# Autodesk Inventor assembly: EmergencyWake
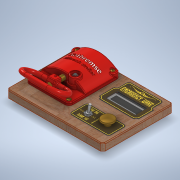
[picture p0: Inventor's stored thumbnail of the model, 180x180]
Saved by Autodesk Inventor 2020 (Build 240168000, 168)
## iProperties
Created: 2020-06-21
Part Number: EmergencyWake
Document SubType Name: Assembly
Designer: Johannes
Author: Johannes
## Documents named in this file (17)
- D:\Dokumente\Projekte\EmergencyWake\CAD\Inventor\EmergencyWake.iam
- D:\Dokumente\Projekte\EmergencyWake\CAD\Inventor\EW_Holzplatte.ipt
- D:\Dokumente\Projekte\EmergencyWake\CAD\Inventor\EW_Display.ipt
- D:\Dokumente\Projekte\EmergencyWake\CAD\Inventor\EW_MessingplatteBedienelemente.ipt
- D:\Dokumente\Projekte\EmergencyWake\CAD\Inventor\EW_MessingplatteUhrzeit.ipt
- D:\Dokumente\Projekte\EmergencyWake\CAD\Inventor\EW_NotbremseGehaeuse.ipt
- D:\Dokumente\Projekte\EmergencyWake\CAD\Inventor\EW_NotbremseHebel.ipt
- D:\Dokumente\Projekte\EmergencyWake\CAD\Inventor\EW_Plexiglas.ipt
- D:\Dokumente\Projekte\EmergencyWake\CAD\Inventor\ToggleSwitchKN3.ipt
- D:\Dokumente\Projekte\EmergencyWake\CAD\Inventor\Board\EmergencyWake.iam
- D:\Dokumente\Projekte\EmergencyWake\CAD\Inventor\DIN964_M5x16_Messing.ipt
- D:\Dokumente\Projekte\EmergencyWake\CAD\Inventor\RotaryEncoder\RotaryEncoder_ALPS_STEC11B.iam
- D:\Dokumente\Projekte\EmergencyWake\CAD\Inventor\EW_Drehknopf.ipt
- D:\Dokumente\Projekte\EmergencyWake\CAD\Inventor\EW_KunststoffEinsatz.ipt
- D:\Dokumente\Projekte\EmergencyWake\CAD\Inventor\EW_HebelAchse.ipt
- D:\Dokumente\Projekte\EmergencyWake\CAD\Inventor\D_090W_06_10mm.ipt
- D:\Dokumente\Projekte\EmergencyWake\CAD\Inventor\EW_Achsenabschluss.ipt
## Components (19 placed, 16 different names)
1. EW_Holzplatte:1 — Passend:1, Passend:2, Passend:3, Fluchtend:1, Fluchtend:2, Fluchtend:3, Fluchtend:4, Fluchtend:5, Passend:5, Passend:6, Fluchtend:6, Passend:8, Passend:9, Passend:10, Passend:11, Passend:12, Winkel:1, Einfügen:6, Winkel:2
2. EW_Display:1 — Passend:7, Fluchtend:7, Fluchtend:8
3. EW_MessingplatteBedienelemente:1 — Passend:2, Fluchtend:5, Passend:4, Einfügen:7
4. EW_MessingplatteUhrzeit:1 — Passend:3, Fluchtend:3, Fluchtend:4, Passend:4
5. EW_NotbremseGehaeuse:1 — Passend:1, Fluchtend:1, Fluchtend:2, Einfügen:2, Einfügen:3, Einfügen:4, Einfügen:5, Einfügen:8, Winkel:3, Winkel:4
6. EW_NotbremseHebel:1 — Einfügen:9, Winkel:4
7. EW_Plexiglas:1 — Passend:5, Passend:6, Fluchtend:6
8. ToggleSwitchKN3:1 — Passend:11, Passend:12, Winkel:1
9. EmergencyWake:1 [sub-assembly] — Passend:7, Fluchtend:7, Fluchtend:8, Passend:8, Passend:9, Passend:10
10. DIN EN ISO 2010 M5x16:1 — Einfügen:2
11. DIN EN ISO 2010 M5x16:2 — Einfügen:3
12. DIN EN ISO 2010 M5x16:3 — Einfügen:5
13. DIN EN ISO 2010 M5x16:4 — Einfügen:4
14. RotaryEncoder_ALPS_STEC11B:1 [sub-assembly] — Einfügen:6, Winkel:2
15. EW_Drehknopf:1 — Einfügen:7
16. EW_KunststoffEinsatz:1 — Einfügen:8, Winkel:3, Passend:13, Passend:14, Passend:16
17. EW_HebelAchse:1 — Passend:13, Passend:14, Einfügen:9, Passend:15, Einfügen:10
18. D_090W_06_10mm:1 — Passend:15, Passend:16
19. EW_Achsenabschluss:1 — Einfügen:10
## Relationships (37: Mate 16, Insert 9, Flush 8, Angle 4)
- Passend:1 [Mate]: EW_Holzplatte:1 ↔ EW_NotbremseGehaeuse:1
- Passend:2 [Mate]: EW_Holzplatte:1 ↔ EW_MessingplatteBedienelemente:1
- Passend:3 [Mate]: EW_Holzplatte:1 ↔ EW_MessingplatteUhrzeit:1
- Fluchtend:1 [Flush] (-10 mm): EW_Holzplatte:1 ↔ EW_NotbremseGehaeuse:1
- Fluchtend:2 [Flush] (-10 mm): EW_Holzplatte:1 ↔ EW_NotbremseGehaeuse:1
- Fluchtend:3 [Flush] (10 mm): EW_Holzplatte:1 ↔ EW_MessingplatteUhrzeit:1
- Fluchtend:4 [Flush] (10 mm): EW_Holzplatte:1 ↔ EW_MessingplatteUhrzeit:1
- Fluchtend:5 [Flush] (10 mm): EW_Holzplatte:1 ↔ EW_MessingplatteBedienelemente:1
- Passend:4 [Mate] (25 mm): EW_MessingplatteBedienelemente:1 ↔ EW_MessingplatteUhrzeit:1
- Passend:5 [Mate]: EW_Holzplatte:1 ↔ EW_Plexiglas:1
- Passend:6 [Mate]: EW_Holzplatte:1 ↔ EW_Plexiglas:1
- Fluchtend:6 [Flush]: EW_Holzplatte:1 ↔ EW_Plexiglas:1
- Passend:7 [Mate] (1 mm): EW_Display:1 ↔ EmergencyWake:1
- Fluchtend:7 [Flush] (0.9 mm): EW_Display:1 ↔ EmergencyWake:1
- Fluchtend:8 [Flush] (10 mm): EW_Display:1 ↔ EmergencyWake:1
- Passend:8 [Mate]: EW_Holzplatte:1 ↔ EmergencyWake:1
- Passend:9 [Mate] (15 mm): EW_Holzplatte:1 ↔ EmergencyWake:1
- Passend:10 [Mate] (2.5 mm): EW_Holzplatte:1 ↔ EmergencyWake:1
- Passend:11 [Mate]: EW_Holzplatte:1 ↔ ToggleSwitchKN3:1
- Passend:12 [Mate]: EW_Holzplatte:1 ↔ ToggleSwitchKN3:1
- Winkel:1 [Angle] (0 deg): EW_Holzplatte:1 ↔ ToggleSwitchKN3:1
- Einfügen:2 [Insert]: EW_NotbremseGehaeuse:1 ↔ DIN EN ISO 2010 M5x16:1
- Einfügen:3 [Insert]: EW_NotbremseGehaeuse:1 ↔ DIN EN ISO 2010 M5x16:2
- Einfügen:4 [Insert]: EW_NotbremseGehaeuse:1 ↔ DIN EN ISO 2010 M5x16:4
- Einfügen:5 [Insert]: EW_NotbremseGehaeuse:1 ↔ DIN EN ISO 2010 M5x16:3
- Einfügen:6 [Insert]: EW_Holzplatte:1 ↔ RotaryEncoder_ALPS_STEC11B:1
- Winkel:2 [Angle] (0 deg): EW_Holzplatte:1 ↔ RotaryEncoder_ALPS_STEC11B:1
- Einfügen:7 [Insert] (1 mm): EW_MessingplatteBedienelemente:1 ↔ EW_Drehknopf:1
- Einfügen:8 [Insert]: EW_NotbremseGehaeuse:1 ↔ EW_KunststoffEinsatz:1
- Winkel:3 [Angle] (0 deg): EW_NotbremseGehaeuse:1 ↔ EW_KunststoffEinsatz:1
- Passend:13 [Mate]: EW_KunststoffEinsatz:1 ↔ EW_HebelAchse:1
- Passend:14 [Mate] (2 mm): EW_KunststoffEinsatz:1 ↔ EW_HebelAchse:1
- Einfügen:9 [Insert]: EW_NotbremseHebel:1 ↔ EW_HebelAchse:1
- Winkel:4 [Angle] (0 deg): EW_NotbremseGehaeuse:1 ↔ EW_NotbremseHebel:1
- Passend:15 [Mate]: EW_HebelAchse:1 ↔ D_090W_06_10mm:1
- Passend:16 [Mate]: EW_KunststoffEinsatz:1 ↔ D_090W_06_10mm:1
- Einfügen:10 [Insert]: EW_HebelAchse:1 ↔ EW_Achsenabschluss:1
